# Autodesk Inventor assembly: measurment ssy
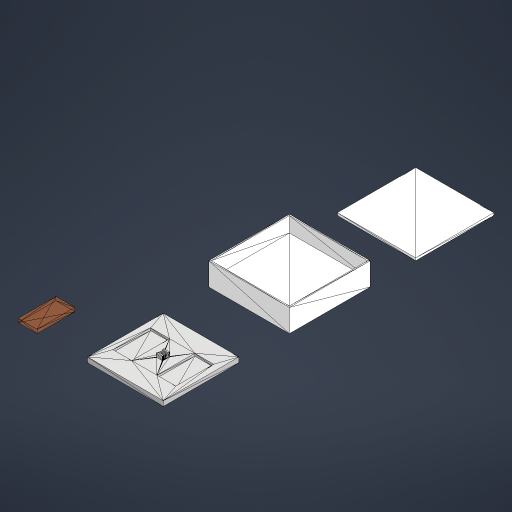
[picture p0: Inventor's stored thumbnail of the model, 512x512]
Saved by Autodesk Inventor 2023 (Build 270158000, 158)
## iProperties
Created: 2023-04-01
Part Number: measurment ssy
Document SubType Name: Assembly
Designer: Jakub
Author: Jakub
## Documents named in this file (5)
- D:\Code\GitHub\VRM_Jakub_Michalica\Project_1\Geometry\measurment ssy.iam
- C:\Users\Jakub\Documents\Inventor\box.ipt
- D:\Code\GitHub\VRM_Jakub_Michalica\Project_1\Geometry\Imported Components\box_cover\box_cover.ipt
- D:\Code\GitHub\VRM_Jakub_Michalica\Project_1\Geometry\Imported Components\carry_frame\carry_frame.ipt
- D:\Code\GitHub\VRM_Jakub_Michalica\Project_1\Geometry\Imported Components\colorblock\colorblock.ipt
## Components (4 placed, 4 different names)
1. box:1 — Flush:4, Flush:5, Flush:6
2. box_cover:1 — Flush:7, Flush:8, Flush:9
3. carry_frame:1 — Flush:1, Flush:2, Flush:3, Flush:4, Flush:5, Flush:6, Flush:7, Flush:8, Flush:9, Flush:10, Flush:11, Flush:12
4. colorblock:1 — Flush:10, Flush:11, Flush:12
## Relationships (12: Flush 12)
- Flush:1: carry_frame:1
- Flush:2: carry_frame:1
- Flush:3: carry_frame:1
- Flush:4: box:1 ↔ carry_frame:1
- Flush:5: box:1 ↔ carry_frame:1
- Flush:6 (5 mm): box:1 ↔ carry_frame:1
- Flush:7: box_cover:1 ↔ carry_frame:1
- Flush:8: box_cover:1 ↔ carry_frame:1
- Flush:9 (10 mm): box_cover:1 ↔ carry_frame:1
- Flush:10: carry_frame:1 ↔ colorblock:1
- Flush:11: carry_frame:1 ↔ colorblock:1
- Flush:12 (5 mm): carry_frame:1 ↔ colorblock:1
